# Autodesk Inventor assembly: forklift_1_0
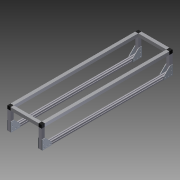
[picture p0: Inventor's stored thumbnail of the model, 180x180]
Saved by Autodesk Inventor 2011 (Build 150239000, 239)
## iProperties
Created: 2013-01-16
Part Number: forklift_1_0
Document SubType Name: Assembly
Designer: 917788
Author: 917788
## Documents named in this file (7)
- F:\Users\Christopher\Documents\GitHub\2013CAD\2013 robot\forklift\frame parts\forklift_1_0.iam
- F:\Users\Christopher\Documents\GitHub\2013CAD\2013 robot\forklift\frame parts\1tube_6.ipt
- F:\Users\Christopher\Documents\GitHub\2013CAD\2013 robot\forklift\frame parts\1tube_9.ipt
- F:\Users\Christopher\Documents\GitHub\2013CAD\2013 robot\forklift\frame parts\1tube_40.ipt
- F:\Users\Christopher\Documents\GitHub\2013CAD\2013 robot\forklift\frame parts\8020_40.ipt
- F:\Users\Christopher\Documents\GitHub\2013CAD\2013 robot\forklift\frame parts\8020_gussetplate.ipt
- F:\Users\Christopher\Documents\GitHub\2013CAD\COTS parts\Plastic_Tubing_Connectors\3-way corner.ipt
## Components (22 placed, 6 different names)
1. 1tube_6:1 — Mate:15, Mate:16, Flush:11, Mate:17, Flush:12, Flush:13, Mate:18, Flush:14, Flush:15, Mate:19, Flush:16, Flush:17
2. 1tube_9:1 — Mate:9, Mate:10, Flush:8, Mate:11, Mate:12, Flush:9
3. 1tube_40:1 — Mate:7, Flush:7, Mate:8, Mate:20, Mate:21, Flush:18
4. 8020_40:1 — Mate:19, Flush:16, Flush:17, Flush:22, Flush:24
5. 8020_gussetplate:1 — Mate:17, Flush:12, Flush:13
6. 1tube_40:2 — Mate:13, Mate:14, Flush:10, Mate:22, Mate:23, Mate:24
7. 1tube_9:2 — Mate:25, Mate:26, Mate:27
8. 1tube_6:2 — Mate:1, Flush:1, Flush:2, Mate:2, Mate:3, Mate:4, Mate:5, Flush:4, Mate:6, Flush:5
9. 8020_40:2 — Mate:1, Flush:1, Flush:2, Flush:3, Flush:6, Flush:20
10. 8020_gussetplate:2 — Mate:36, Flush:23, Flush:24
11. 8020_gussetplate:3 — Mate:18, Flush:14, Flush:15
12. 8020_gussetplate:4 — Mate:6, Flush:5, Flush:6
13. 8020_gussetplate:5 — Mate:5, Flush:3, Flush:4
14. 8020_gussetplate:7 — Mate:35, Flush:21, Flush:22
15. 8020_gussetplate:8 — Mate:31, Flush:19, Flush:20
16. 8020_gussetplate:9 — Mate:37, Flush:25, Flush:26
17. 3-way corner:1 — Mate:11, Mate:12, Flush:9, Mate:13, Mate:14, Flush:10, Mate:15, Mate:16, Flush:11
18. 3-way corner:2 — Mate:2, Mate:3, Mate:4, Mate:7, Flush:7, Mate:8, Mate:9, Mate:10, Flush:8
19. 3-way corner:3 — Mate:20, Mate:21, Flush:18, Mate:25, Mate:28, Mate:29, Mate:30
20. 3-way corner:4 — Mate:22, Mate:23, Mate:24, Mate:26, Mate:27, Mate:32, Mate:33, Mate:34
21. 1tube_6:3 — Mate:32, Mate:33, Mate:34, Mate:35, Flush:21, Mate:36, Flush:23
22. 1tube_6:4 — Mate:28, Mate:29, Mate:30, Mate:31, Flush:19, Mate:37, Flush:25, Flush:26
## Relationships (63: Mate 37, Flush 26)
- Mate:1: 1tube_6:2 ↔ 8020_40:2
- Flush:1: 1tube_6:2 ↔ 8020_40:2
- Flush:2: 1tube_6:2 ↔ 8020_40:2
- Mate:2: 1tube_6:2 ↔ 3-way corner:2
- Mate:3: 1tube_6:2 ↔ 3-way corner:2
- Mate:4: 1tube_6:2 ↔ 3-way corner:2
- Mate:5: 1tube_6:2 ↔ 8020_gussetplate:5
- Flush:3: 8020_40:2 ↔ 8020_gussetplate:5
- Flush:4: 1tube_6:2 ↔ 8020_gussetplate:5
- Mate:6: 1tube_6:2 ↔ 8020_gussetplate:4
- Flush:5: 1tube_6:2 ↔ 8020_gussetplate:4
- Flush:6: 8020_40:2 ↔ 8020_gussetplate:4
- Mate:7: 1tube_40:1 ↔ 3-way corner:2
- Flush:7: 1tube_40:1 ↔ 3-way corner:2
- Mate:8: 1tube_40:1 ↔ 3-way corner:2
- Mate:9: 1tube_9:1 ↔ 3-way corner:2
- Mate:10: 1tube_9:1 ↔ 3-way corner:2
- Flush:8: 1tube_9:1 ↔ 3-way corner:2
- Mate:11: 1tube_9:1 ↔ 3-way corner:1
- Mate:12: 1tube_9:1 ↔ 3-way corner:1
- Flush:9: 1tube_9:1 ↔ 3-way corner:1
- Mate:13: 1tube_40:2 ↔ 3-way corner:1
- Mate:14: 1tube_40:2 ↔ 3-way corner:1
- Flush:10: 1tube_40:2 ↔ 3-way corner:1
- Mate:15: 1tube_6:1 ↔ 3-way corner:1
- Mate:16: 1tube_6:1 ↔ 3-way corner:1
- Flush:11: 1tube_6:1 ↔ 3-way corner:1
- Mate:17: 1tube_6:1 ↔ 8020_gussetplate:1
- Flush:12: 1tube_6:1 ↔ 8020_gussetplate:1
- Flush:13: 1tube_6:1 ↔ 8020_gussetplate:1
- Mate:18: 1tube_6:1 ↔ 8020_gussetplate:3
- Flush:14: 1tube_6:1 ↔ 8020_gussetplate:3
- Flush:15: 1tube_6:1 ↔ 8020_gussetplate:3
- Mate:19: 1tube_6:1 ↔ 8020_40:1
- Flush:16: 1tube_6:1 ↔ 8020_40:1
- Flush:17: 1tube_6:1 ↔ 8020_40:1
- Mate:20: 1tube_40:1 ↔ 3-way corner:3
- Mate:21: 1tube_40:1 ↔ 3-way corner:3
- Flush:18: 1tube_40:1 ↔ 3-way corner:3
- Mate:22: 1tube_40:2 ↔ 3-way corner:4
- Mate:23: 1tube_40:2 ↔ 3-way corner:4
- Mate:24: 1tube_40:2 ↔ 3-way corner:4
- Mate:25: 1tube_9:2 ↔ 3-way corner:3
- Mate:26: 1tube_9:2 ↔ 3-way corner:4
- Mate:27: 1tube_9:2 ↔ 3-way corner:4
- Mate:28: 3-way corner:3 ↔ 1tube_6:4
- Mate:29: 3-way corner:3 ↔ 1tube_6:4
- Mate:30: 3-way corner:3 ↔ 1tube_6:4
- Mate:31: 8020_gussetplate:8 ↔ 1tube_6:4
- Flush:19: 8020_gussetplate:8 ↔ 1tube_6:4
- Flush:20: 8020_40:2 ↔ 8020_gussetplate:8
- Mate:32: 3-way corner:4 ↔ 1tube_6:3
- Mate:33: 3-way corner:4 ↔ 1tube_6:3
- Mate:34: 3-way corner:4 ↔ 1tube_6:3
- Mate:35: 8020_gussetplate:7 ↔ 1tube_6:3
- Flush:21: 8020_gussetplate:7 ↔ 1tube_6:3
- Flush:22: 8020_40:1 ↔ 8020_gussetplate:7
- Mate:36: 8020_gussetplate:2 ↔ 1tube_6:3
- Flush:23: 8020_gussetplate:2 ↔ 1tube_6:3
- Flush:24: 8020_40:1 ↔ 8020_gussetplate:2
- Mate:37: 8020_gussetplate:9 ↔ 1tube_6:4
- Flush:25: 8020_gussetplate:9 ↔ 1tube_6:4
- Flush:26: 8020_gussetplate:9 ↔ 1tube_6:4
